# Autodesk Inventor assembly: ForeArm
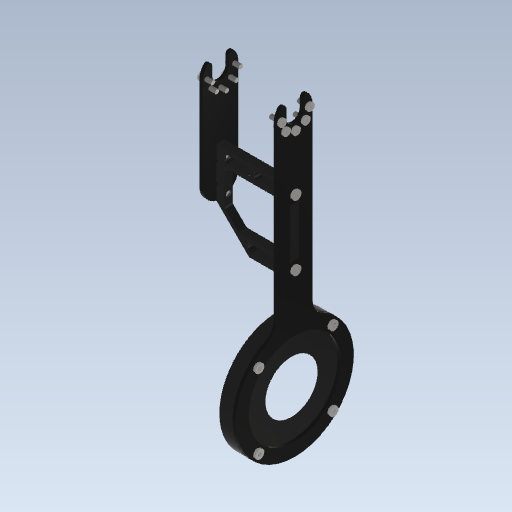
[picture p0: Inventor's stored thumbnail of the model, 512x512]
Saved by Autodesk Inventor 2020.4 (Build 244396000, 396)
## iProperties
Created: 2022-01-10
Part Number: ForeArm
Document SubType Name: Assembly
Designer: Masato Kubotera
Author: Masato Kubotera
## Documents named in this file (9)
- C:\Users\Masato\Documents\Inventor\CIT Brains_Inventor\OpenPlatform_ver3_0\UpperBody\Arm\ForeArm.iam
- C:\Users\Masato\Documents\Inventor\CIT Brains_Inventor\OpenPlatform_ver3_0\UpperBody\Arm\ForeArm_outside_frame.ipt
- C:\Users\Masato\Documents\Inventor\CIT Brains_Inventor\OpenPlatform_ver3_0\UpperBody\Arm\ForeArm_hand.ipt
- C:\Users\Masato\Documents\Inventor\CIT Brains_Inventor\OpenPlatform_ver3_0\UpperBody\Arm\ForeArm_inside_frame.ipt
- C:\Users\Masato\Documents\Inventor\CIT Brains_Inventor\OpenPlatform_ver3_0\ReadyMade\InsertNut\UD-43040.ipt
- C:\Users\Masato\Documents\Inventor\CIT Brains_Inventor\OpenPlatform_ver3_0\ReadyMade\Screw\M3-6.ipt
- C:\Users\Masato\Documents\Inventor\CIT Brains_Inventor\OpenPlatform_ver3_0\ReadyMade\Screw\M2_6-6.ipt
- C:\Users\Masato\Documents\Inventor\CIT Brains_Inventor\OpenPlatform_ver3_0\ReadyMade\InsertNut\IRU-304SW.ipt
- C:\Users\Masato\Documents\Inventor\CIT Brains_Inventor\OpenPlatform_ver3_0\UpperBody\Arm\ForeArm_diagonal.ipt
## Components (30 placed, 8 different names)
1. ForeArm_outside_frame:1 — 挿入:7, 挿入:9, 挿入:10, 挿入:15, 挿入:16, 挿入:17, 挿入:18, 挿入:23, 挿入:24, 挿入:27, 挿入:28, 挿入:31, 挿入:32, 挿入:33, 挿入:34, メイト:1, メイト:2, フラッシュ:1, 挿入:8, 挿入:39
2. ForeArm_hand:1 — 挿入:1, 挿入:2, 挿入:3, 挿入:4, 挿入:8
3. ForeArm_inside_frame:1 — 挿入:25, 挿入:26, 挿入:29, 挿入:30, 挿入:35, 挿入:36, 挿入:37, 挿入:38, 挿入:40
4. ForeArm_diagonal:1 — 挿入:19, 挿入:20, 挿入:21, 挿入:22
5. M2_6-6:9 — 挿入:39
6. M2_6-6:10 — 挿入:40
7. M3-6:10 — 挿入:30
8. M3-6:9 — 挿入:29
9. M3-6:8 — 挿入:28
10. M3-6:7 — 挿入:27
11. M2_6-6:8 — 挿入:38
12. M2_6-6:7 — 挿入:37
13. M2_6-6:6 — 挿入:36
14. M2_6-6:5 — 挿入:35
15. M2_6-6:4 — 挿入:34
16. M2_6-6:3 — 挿入:33
17. M2_6-6:2 — 挿入:32
18. M2_6-6:1 — 挿入:31
19. M3-6:6 — 挿入:18
20. M3-6:5 — 挿入:17
21. M3-6:4 — 挿入:16
22. M3-6:3 — 挿入:15
23. UD-43040:4 — 挿入:4, 挿入:10
24. UD-43040:3 — 挿入:3, 挿入:9
25. UD-43040:2 — 挿入:2
26. UD-43040:1 — 挿入:1, 挿入:7
27. IRU-304SW:1 — 挿入:19, 挿入:23
28. IRU-304SW:2 — 挿入:20, 挿入:24
29. IRU-304SW:3 — 挿入:21, 挿入:25
30. IRU-304SW:4 — 挿入:22, 挿入:26
## Relationships (37: Insert 34, Mate 2, Flush 1)
- 挿入:1 [Insert]: ForeArm_hand:1 ↔ UD-43040:1
- 挿入:2 [Insert]: ForeArm_hand:1 ↔ UD-43040:2
- 挿入:3 [Insert]: ForeArm_hand:1 ↔ UD-43040:3
- 挿入:4 [Insert]: ForeArm_hand:1 ↔ UD-43040:4
- 挿入:7 [Insert]: ForeArm_outside_frame:1 ↔ UD-43040:1
- 挿入:8 [Insert]: ForeArm_outside_frame:1 ↔ ForeArm_hand:1
- 挿入:9 [Insert]: ForeArm_outside_frame:1 ↔ UD-43040:3
- 挿入:10 [Insert]: ForeArm_outside_frame:1 ↔ UD-43040:4
- 挿入:15 [Insert]: ForeArm_outside_frame:1 ↔ M3-6:3
- 挿入:16 [Insert]: ForeArm_outside_frame:1 ↔ M3-6:4
- 挿入:17 [Insert]: ForeArm_outside_frame:1 ↔ M3-6:5
- 挿入:18 [Insert]: ForeArm_outside_frame:1 ↔ M3-6:6
- 挿入:19 [Insert]: ForeArm_diagonal:1 ↔ IRU-304SW:1
- 挿入:20 [Insert]: ForeArm_diagonal:1 ↔ IRU-304SW:2
- 挿入:21 [Insert]: ForeArm_diagonal:1 ↔ IRU-304SW:3
- 挿入:22 [Insert]: ForeArm_diagonal:1 ↔ IRU-304SW:4
- 挿入:23 [Insert]: ForeArm_outside_frame:1 ↔ IRU-304SW:1
- 挿入:24 [Insert]: ForeArm_outside_frame:1 ↔ IRU-304SW:2
- 挿入:25 [Insert]: ForeArm_inside_frame:1 ↔ IRU-304SW:3
- 挿入:26 [Insert]: ForeArm_inside_frame:1 ↔ IRU-304SW:4
- 挿入:27 [Insert]: ForeArm_outside_frame:1 ↔ M3-6:7
- 挿入:28 [Insert]: ForeArm_outside_frame:1 ↔ M3-6:8
- 挿入:29 [Insert]: ForeArm_inside_frame:1 ↔ M3-6:9
- 挿入:30 [Insert]: ForeArm_inside_frame:1 ↔ M3-6:10
- 挿入:31 [Insert]: ForeArm_outside_frame:1 ↔ M2_6-6:1
- 挿入:32 [Insert]: ForeArm_outside_frame:1 ↔ M2_6-6:2
- 挿入:33 [Insert]: ForeArm_outside_frame:1 ↔ M2_6-6:3
- 挿入:34 [Insert]: ForeArm_outside_frame:1 ↔ M2_6-6:4
- 挿入:35 [Insert]: ForeArm_inside_frame:1 ↔ M2_6-6:5
- 挿入:36 [Insert]: ForeArm_inside_frame:1 ↔ M2_6-6:6
- 挿入:37 [Insert]: ForeArm_inside_frame:1 ↔ M2_6-6:7
- 挿入:38 [Insert]: ForeArm_inside_frame:1 ↔ M2_6-6:8
- メイト:1 [Mate]: ForeArm_outside_frame:1
- メイト:2 [Mate]: ForeArm_outside_frame:1
- フラッシュ:1 [Flush]: ForeArm_outside_frame:1
- 挿入:39 [Insert]: ForeArm_outside_frame:1 ↔ M2_6-6:9
- 挿入:40 [Insert]: ForeArm_inside_frame:1 ↔ M2_6-6:10
